# Autodesk Inventor assembly: plane_assembly
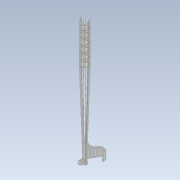
[picture p0: Inventor's stored thumbnail of the model, 180x180]
Saved by Autodesk Inventor 2020 (Build 240168000, 168)
## iProperties
Created: 2020-09-10
Part Number: plane_assembly
Document SubType Name: Assembly
Designer: Admin
Author: Admin
## Documents named in this file (5)
- C:\PFE\Project_github\YFA-Project_python_interface\3D models\plane_assembly.iam
- C:\PFE\Project_github\YFA-Project_python_interface\3D models\traverse_cote - top.ipt
- C:\PFE\Project_github\YFA-Project_python_interface\3D models\traverse_cote.ipt
- C:\PFE\Project_github\YFA-Project_python_interface\3D models\traverse_cote - bottom.ipt
- C:\PFE\Project_github\YFA-Project_python_interface\3D models\main_ring.ipt
## Components (12 placed, 4 different names)
1. traverse_cote - top:1 — Angle:1, Angle:2, Angle:3, Angle:4, Angle:5, Mate:13, Mate:14, Mate:15, Mate:20, Mate:26, Mate:30, Mate:31, Mate:32, Mate:33
2. traverse_cote:1 — Angle:1, Mate:3, Mate:4, Mate:5
3. traverse_cote:2 — Angle:2, Mate:7, Mate:8, Mate:9
4. traverse_cote:3 — Angle:3, Mate:10, Mate:11, Mate:12
5. traverse_cote:4 — Angle:4, Mate:16, Mate:17, Mate:18, Mate:27, Mate:28, Mate:29
6. traverse_cote - bottom:1 — Angle:5, Mate:1, Mate:2, Mate:6, Mate:19
7. main_ring:1 — Mate:1, Mate:2, Mate:3, Mate:4, Mate:5, Mate:6, Mate:7, Mate:8, Mate:9, Mate:10, Mate:11, Mate:12, Mate:13, Mate:14, Mate:15, Mate:16, Mate:17, Mate:18, Mate:21, Flush:1
8. main_ring:2 — Mate:19, Mate:20, Mate:21, Mate:22, Mate:32
9. main_ring:3 — Mate:25, Mate:26, Flush:1
10. main_ring:4 — Mate:24, Mate:25, Mate:27, Mate:30
11. main_ring:5 — Mate:22, Mate:23, Mate:28, Mate:31
12. main_ring:6 — Mate:23, Mate:24, Mate:29, Mate:33
## Relationships (39: Mate 33, Angle 5, Flush 1)
- Angle:1 (60 deg): traverse_cote - top:1 ↔ traverse_cote:1
- Angle:2 (60 deg): traverse_cote - top:1 ↔ traverse_cote:2
- Angle:3 (120 deg): traverse_cote - top:1 ↔ traverse_cote:3
- Angle:4 (-120 deg): traverse_cote - top:1 ↔ traverse_cote:4
- Angle:5 (0 deg): traverse_cote - top:1 ↔ traverse_cote - bottom:1
- Mate:1: traverse_cote - bottom:1 ↔ main_ring:1
- Mate:2: traverse_cote - bottom:1 ↔ main_ring:1
- Mate:3: traverse_cote:1 ↔ main_ring:1
- Mate:4: traverse_cote:1 ↔ main_ring:1
- Mate:5: traverse_cote:1 ↔ main_ring:1
- Mate:6: traverse_cote - bottom:1 ↔ main_ring:1
- Mate:7: traverse_cote:2 ↔ main_ring:1
- Mate:8: traverse_cote:2 ↔ main_ring:1
- Mate:9: traverse_cote:2 ↔ main_ring:1
- Mate:10: traverse_cote:3 ↔ main_ring:1
- Mate:11: traverse_cote:3 ↔ main_ring:1
- Mate:12: traverse_cote:3 ↔ main_ring:1
- Mate:13: traverse_cote - top:1 ↔ main_ring:1
- Mate:14: traverse_cote - top:1 ↔ main_ring:1
- Mate:15: traverse_cote - top:1 ↔ main_ring:1
- Mate:16: traverse_cote:4 ↔ main_ring:1
- Mate:17: traverse_cote:4 ↔ main_ring:1
- Mate:18: traverse_cote:4 ↔ main_ring:1
- Mate:19: traverse_cote - bottom:1 ↔ main_ring:2
- Mate:20: traverse_cote - top:1 ↔ main_ring:2
- Mate:21: main_ring:1 ↔ main_ring:2
- Mate:22: main_ring:2 ↔ main_ring:5
- Mate:23: main_ring:5 ↔ main_ring:6
- Mate:24: main_ring:4 ↔ main_ring:6
- Mate:25: main_ring:3 ↔ main_ring:4
- Mate:26: traverse_cote - top:1 ↔ main_ring:3
- Mate:27: traverse_cote:4 ↔ main_ring:4
- Mate:28: traverse_cote:4 ↔ main_ring:5
- Mate:29: traverse_cote:4 ↔ main_ring:6
- Flush:1 (40 mm): main_ring:1 ↔ main_ring:3
- Mate:30: traverse_cote - top:1 ↔ main_ring:4
- Mate:31: traverse_cote - top:1 ↔ main_ring:5
- Mate:32: traverse_cote - top:1 ↔ main_ring:2
- Mate:33: traverse_cote - top:1 ↔ main_ring:6
